# Autodesk Inventor assembly: Femto
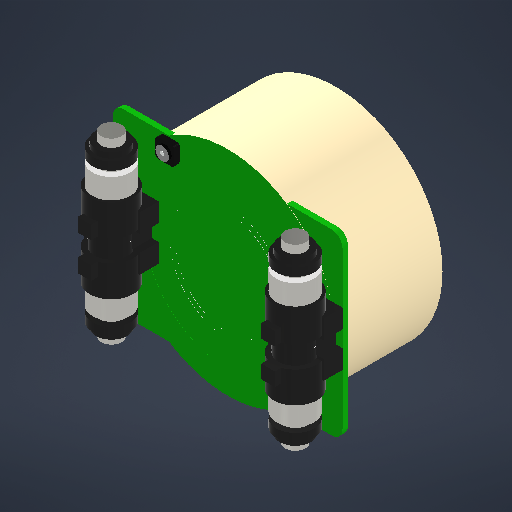
[picture p0: Inventor's stored thumbnail of the model, 512x512]
Saved by Autodesk Inventor 2026.1 (Build 301233000, 233)
## iProperties
Created: 2025-11-06
Part Number: Femto
Document SubType Name: Assembly
Designer: SPEL
Author: SPEL
## Documents named in this file (3)
- C:\Users\SPEL\Desktop\SPEL\Femto\Femto.iam
- C:\Users\SPEL\Desktop\SPEL\Femto\PCB.ipt
- C:\Users\SPEL\Desktop\SPEL\Femto\injector femto.ipt
## Components (5 placed, 2 different names)
1. PCB:1 — Flush:1, Flush:2, Flush:3, Flush:4, Mate:1, Mate:2, Mate:3, Mate:4, Flush:5, Flush:6, Flush:7, Flush:8
2. injector femto:1 — Flush:1, Mate:3, Flush:5
3. injector femto:2 — Flush:2, Mate:1, Flush:7
4. injector femto:3 — Flush:4, Mate:2, Flush:8
5. injector femto:4 — Flush:3, Mate:4, Flush:6
## Relationships (12: Flush 8, Mate 4)
- Flush:1: PCB:1 ↔ injector femto:1
- Flush:2: PCB:1 ↔ injector femto:2
- Flush:3: PCB:1 ↔ injector femto:4
- Flush:4: PCB:1 ↔ injector femto:3
- Mate:1: PCB:1 ↔ injector femto:2
- Mate:2: PCB:1 ↔ injector femto:3
- Mate:3: PCB:1 ↔ injector femto:1
- Mate:4: PCB:1 ↔ injector femto:4
- Flush:5: PCB:1 ↔ injector femto:1
- Flush:6: PCB:1 ↔ injector femto:4
- Flush:7: PCB:1 ↔ injector femto:2
- Flush:8: PCB:1 ↔ injector femto:3
